# Autodesk Inventor assembly: lemon shape asse
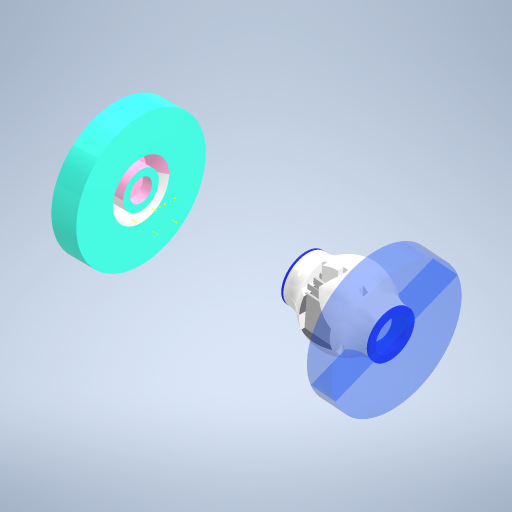
[picture p0: Inventor's stored thumbnail of the model, 512x512]
Saved by Autodesk Inventor 2023 (Build 270158000, 158)
## iProperties
Created: 2022-11-14
Part Number: lemon shape asse
Document SubType Name: Assembly
Designer: RM206user
Author: RM206user
## Documents named in this file (10)
- C:\Users\RM206user\Desktop\cansat\tanekonsat2022_runback\machinary\parts\tire\lemon shape asse.iam
- C:\Users\RM206user\Desktop\cansat\tanekonsat2022_runback\machinary\parts\tire\130 25 lemon tire.iam
- C:\Users\RM206user\Desktop\cansat\tanekonsat2022_runback\machinary\parts\bush.ipt
- C:\Users\RM206user\Desktop\cansat\tanekonsat2022_runback\machinary\body\body back\back moter middle tire ver\back moter middle tire lemon shape.ipt
- C:\Users\RM206user\Desktop\cansat\tanekonsat2022_runback\machinary\body\body front\front moter middle basic\body front moter middle lemon shape.ipt
- C:\Users\RM206user\Desktop\cansat\tanekonsat2022_runback\machinary\body\body back\back for main connection\body back for main 3.ipt
- C:\Users\RM206user\Desktop\cansat\tanekonsat2022_runback\machinary\parts\GNSS1.ipt
- C:\Users\RM206user\Desktop\cansat\tanekonsat2022_runback\machinary\parts\almi1.ipt
- C:\Users\RM206user\Desktop\cansat\tanekonsat2022_runback\machinary\parts\almi2.ipt
- C:\Users\RM206user\Desktop\cansat\tanekonsat2022_runback\machinary\parts\mein1.ipt
## Components (11 placed, 9 different names)
1. 130 25 lemon tire:1 [sub-assembly]
2. 130 25 lemon tire:2 [sub-assembly] — メイト:24, メイト:25
3. bush:1 — メイト:22, メイト:23
4. bush:2 — メイト:20, メイト:21, メイト:24, メイト:25
5. body moter middle:1 — メイト:1, メイト:2, メイト:12, メイト:18, メイト:19, メイト:20
6. base front:1 — メイト:3, メイト:4, メイト:5, メイト:6, メイト:7, メイト:8, メイト:9, メイト:12, メイト:13, メイト:14, メイト:15, メイト:16, メイト:17, メイト:18, メイト:19, メイト:21, メイト:22, メイト:23
7. body back:1 — メイト:1, メイト:2
8. GNSS1:1 — メイト:13, メイト:14, メイト:15
9. almi1:1 — メイト:6, メイト:7, メイト:16
10. almi2:1 — メイト:3, メイト:4, メイト:5
11. mein1:1 — メイト:8, メイト:9, メイト:17
## Relationships (23: Mate 23)
- メイト:1 [Mate]: body moter middle:1 ↔ body back:1
- メイト:2 [Mate]: body moter middle:1 ↔ body back:1
- メイト:3 [Mate]: base front:1 ↔ almi2:1
- メイト:4 [Mate]: base front:1 ↔ almi2:1
- メイト:5 [Mate]: base front:1 ↔ almi2:1
- メイト:6 [Mate]: base front:1 ↔ almi1:1
- メイト:7 [Mate]: base front:1 ↔ almi1:1
- メイト:8 [Mate]: base front:1 ↔ mein1:1
- メイト:9 [Mate]: base front:1 ↔ mein1:1
- メイト:12 [Mate]: body moter middle:1 ↔ base front:1
- メイト:13 [Mate]: base front:1 ↔ GNSS1:1
- メイト:14 [Mate]: base front:1 ↔ GNSS1:1
- メイト:15 [Mate]: base front:1 ↔ GNSS1:1
- メイト:16 [Mate]: base front:1 ↔ almi1:1
- メイト:17 [Mate]: base front:1 ↔ mein1:1
- メイト:18 [Mate]: body moter middle:1 ↔ base front:1
- メイト:19 [Mate]: body moter middle:1 ↔ base front:1
- メイト:20 [Mate]: bush:2 ↔ body moter middle:1
- メイト:21 [Mate]: bush:2 ↔ base front:1
- メイト:22 [Mate]: bush:1 ↔ base front:1
- メイト:23 [Mate]: bush:1 ↔ base front:1
- メイト:24 [Mate]: 130 25 lemon tire:2 ↔ bush:2
- メイト:25 [Mate] (-20 mm): 130 25 lemon tire:2 ↔ bush:2
